# Autodesk Inventor assembly: am-940a-6-HiGrip-_MIR2
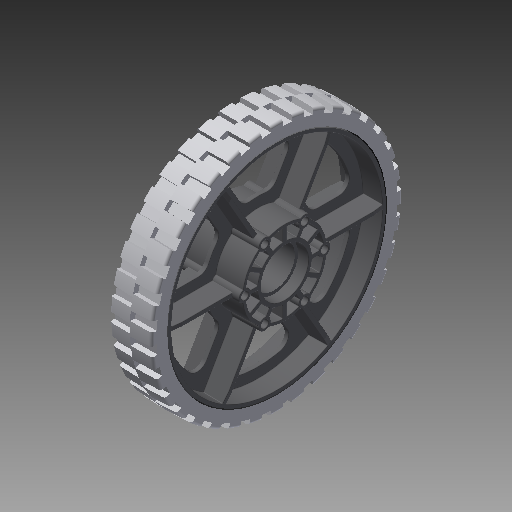
[picture p0: Inventor's stored thumbnail of the model, 512x512]
Saved by Autodesk Inventor 2018.2 (Build 222227000, 227)
## iProperties
Created: 2014-03-19
Part Number: am-940a-6-HiGrip-_MIR2
Description: STEP AP214
Document SubType Name: Assembly
Designer: steele
Title: 6-HiGrip-am-940aSTEP.STEP
Revision Number: ANY
Sending System: SolidWorks 2010
Preprocessor: SwSTEP 2.0
## Documents named in this file (3)
- D:\snobotics\CAD-Development\robSteele\SnoBotics2016\2016-01-23-BallShooter\am-940a-6-HiGrip-_MIR2.iam
- D:\snobotics\CAD-Development\robSteele\SnoBotics2016\2016-01-23-BallShooter\6 wheel Rev 4_MIR2.ipt
- D:\snobotics\CAD-Development\robSteele\SnoBotics2016\2016-01-23-BallShooter\6 wheel tread II_MIR2.ipt
## Components (2 placed, 2 different names)
1. 6 wheel Rev 4_MIR2:1
2. 6 wheel tread II_MIR2:1 — Flush:1
## Relationships (1: Flush 1)
- Flush:1 (-12.7 mm): 6 wheel tread II_MIR2:1
